# Autodesk Inventor assembly: Marco_apm_001-3
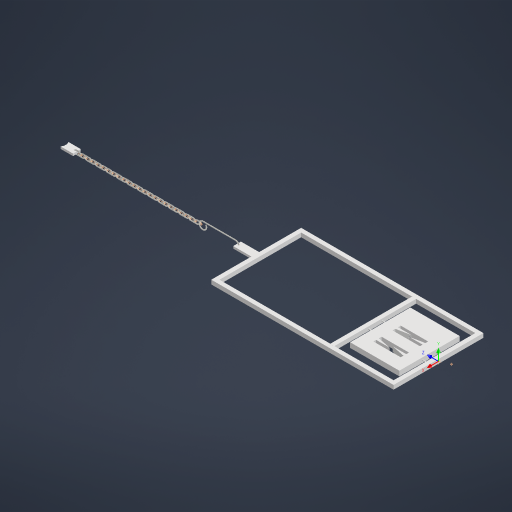
[picture p0: Inventor's stored thumbnail of the model, 512x512]
Saved by Autodesk Inventor 2024 (Build 280153000, 153)
## iProperties
Created: 2023-05-17
Part Number: Marco_apm_001-3
Document SubType Name: Assembly
Designer: javie
Author: javie
## Documents named in this file (6)
- C:\Users\javie\Downloads\Piezas CMR\Marco_APM_001\Marco_apm_001-3.iam
- C:\Users\javie\Downloads\Piezas CMR\Marco_Conveyor_Aereo.iam
- C:\Users\javie\Downloads\Piezas CMR\Marcos_solids\Topes_apm_002-2.ipt
- C:\Users\javie\Downloads\Piezas CMR\Marcos_solids\S_horizontal.ipt
- C:\Users\javie\Downloads\Piezas CMR\Marco_APM_001\Partes\APM_001-3.ipt
- C:\Users\javie\Downloads\Piezas CMR\Marcos_solids\0010.ipt
## Components (6 placed, 5 different names)
1. Marco_Conveyor_Aereo:1 [sub-assembly] — Insertar:8, Nivelación:1, Nivelación:2
2. Topes_apm_002-2:1 — Insertar:3, Insertar:11, Insertar:12
3. S_horizontal:1 — Insertar:3
4. APM_001-3:1 — Insertar:9, Insertar:10, Insertar:11, Insertar:12
5. Topes_apm_002-2:2 — Insertar:8, Insertar:9, Insertar:10
6. 0010:1 — Nivelación:1, Nivelación:2
## Relationships (8: Insert 6, Flush 2)
- Insertar:3: Topes_apm_002-2:1 ↔ S_horizontal:1
- Insertar:8: Marco_Conveyor_Aereo:1 ↔ Topes_apm_002-2:2
- Insertar:9: APM_001-3:1 ↔ Topes_apm_002-2:2
- Insertar:10: APM_001-3:1 ↔ Topes_apm_002-2:2
- Insertar:11: Topes_apm_002-2:1 ↔ APM_001-3:1
- Insertar:12: Topes_apm_002-2:1 ↔ APM_001-3:1
- Nivelación:1 [Flush]: Marco_Conveyor_Aereo:1 ↔ 0010:1
- Nivelación:2 [Flush]: Marco_Conveyor_Aereo:1 ↔ 0010:1
